# Autodesk Inventor assembly: Correct
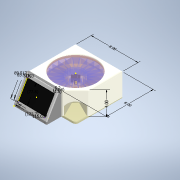
[picture p0: Inventor's stored thumbnail of the model, 180x180]
Saved by Autodesk Inventor 2022 (Build 260153000, 153)
## iProperties
Created: 2023-02-27
Part Number: Correct
Document SubType Name: Assembly
Designer: zarek
Author: zarek
## Documents named in this file (12)
- C:\Users\zarek\OneDrive\Desktop\Random New Stuff\SPB\Correct.iam
- C:\Users\zarek\OneDrive\Desktop\Random New Stuff\SPB\Base_Plate_2.ipt
- C:\Users\zarek\OneDrive\Desktop\Random New Stuff\SPB\Capsule_Design_Final.ipt
- C:\Users\zarek\OneDrive\Desktop\Random New Stuff\SPB\Motor_Key.ipt
- C:\Users\zarek\OneDrive\Desktop\Random New Stuff\SPB\GrabCad Parts\Stepper 28BYJ48.ipt
- C:\Users\zarek\OneDrive\Desktop\Random New Stuff\SPB\Drop_Plate.ipt
- C:\Users\zarek\OneDrive\Desktop\Random New Stuff\SPB\Box_Walls_2.ipt
- C:\Users\zarek\OneDrive\Desktop\Random New Stuff\SPB\Lid Parts\Lid Assembly.iam
- C:\Users\zarek\OneDrive\Desktop\Random New Stuff\SPB\Servo&Holder.iam
- C:\Users\zarek\OneDrive\Desktop\Random New Stuff\SPB\Hook.ipt
- C:\Users\zarek\OneDrive\Desktop\Random New Stuff\SPB\Lid_Inside_Base.ipt
- C:\Users\zarek\OneDrive\Desktop\Random New Stuff\SPB\TouchScreen Housing\Touch Screen Assembly_2.iam
## Components (11 placed, 11 different names)
1. Base_Plate_2:1 — Slider:1, Flush:1, Mate:3, Flush:2, Flush:3, Mate:5, Mate:6, Mate:7
2. Capsule_Design_Final:1 — Rotational:2
3. Motor_Key:1 — Rotational:1, Rotational:2
4. Stepper 28BYJ48:1 — Slider:1, Rotational:1
5. Drop_Plate:1 — Mate:5, Mate:6, Mate:7
6. Box_Walls_2:1 — Flush:1, Mate:3, Flush:2, Flush:3, Slider:2
7. Lid Assembly:1 [sub-assembly] — Slider:2
8. Servo&Holder:1 [sub-assembly] — Rotational:3
9. Hook:1 — Rotational:3
10. Lid_Inside_Base:1
11. Touch Screen Assembly_2:1 [sub-assembly]
## Relationships (12: Mate 4, RevoluteJoint 3, Flush 3, TranslationJoint 2)
- Slider:1 [TranslationJoint]: Base_Plate_2:1 ↔ Stepper 28BYJ48:1
- Rotational:1 [RevoluteJoint]: Motor_Key:1 ↔ Stepper 28BYJ48:1
- Flush:1: Base_Plate_2:1 ↔ Box_Walls_2:1
- Mate:3: Base_Plate_2:1 ↔ Box_Walls_2:1
- Flush:2: Base_Plate_2:1 ↔ Box_Walls_2:1
- Flush:3: Base_Plate_2:1 ↔ Box_Walls_2:1
- Mate:5: Base_Plate_2:1 ↔ Drop_Plate:1
- Mate:6: Base_Plate_2:1 ↔ Drop_Plate:1
- Rotational:2 [RevoluteJoint] (1 mm): Capsule_Design_Final:1 ↔ Motor_Key:1
- Slider:2 [TranslationJoint]: Box_Walls_2:1 ↔ Lid Assembly:1
- Rotational:3 [RevoluteJoint]: Servo&Holder:1 ↔ Hook:1
- Mate:7: Base_Plate_2:1 ↔ Drop_Plate:1
